# Autodesk Inventor assembly: Втулка+косозубка-мини
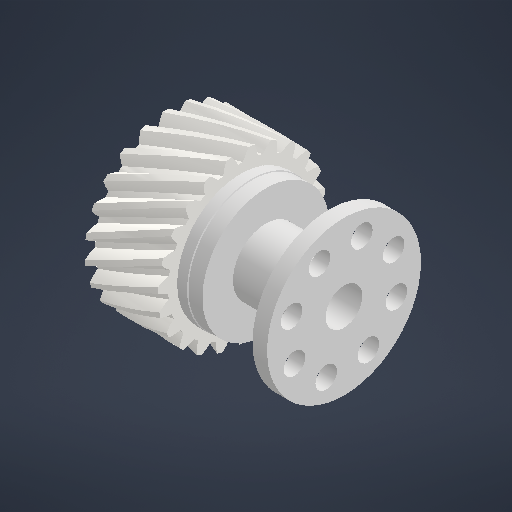
[picture p0: Inventor's stored thumbnail of the model, 512x512]
Saved by Autodesk Inventor 2025 (Build 290162000, 162)
## iProperties
Created: 2025-09-25
Part Number: Втулка+косозубка-мини
Document SubType Name: Assembly
Designer: Phantom
Author: Phantom
## Documents named in this file (3)
- C:\Users\Phantom\Desktop\Phantom16950\Работы Arty\Втулка+косозубка-мини.iam
- C:\Users\Phantom\Desktop\Phantom16950\звезда и втулка.iam
- C:\Users\Phantom\Desktop\Phantom16950\Работы Arty\Косозубая Малая АРКА.ipt
## Components (2 placed, 2 different names)
1. звезда и втулка:1 [sub-assembly] — Цилиндрический:1, Заподлицо:1
2. Цилиндрическое зубчатое зацепление1:1 — Цилиндрический:1, Заподлицо:1
## Relationships (2: CylindricalJoint 1, Flush 1)
- Цилиндрический:1 [CylindricalJoint]: звезда и втулка:1 ↔ Цилиндрическое зубчатое зацепление1:1
- Заподлицо:1 [Flush]: звезда и втулка:1 ↔ Цилиндрическое зубчатое зацепление1:1
